# Autodesk Inventor assembly: ETrigger
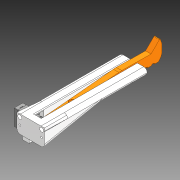
[picture p0: Inventor's stored thumbnail of the model, 180x180]
Saved by Autodesk Inventor 2020 (Build 240168000, 168)
## iProperties
Created: 2020-09-14
Part Number: ETrigger
Document SubType Name: Assembly
Designer: DDeGo
Author: DDeGo
Revision Number: PRODUCT_VERSION_IDPRODUCT_VERSION_DESCR
## Documents named in this file (4)
- C:\Users\DDeGo\Documents\Drew\Projects\Nerf Aim Assist\ESPER\ETrigger.iam
- C:\Users\DDeGo\Documents\Drew\Projects\Nerf Aim Assist\ESPER\SearE.ipt
- C:\Users\DDeGo\Documents\Drew\Projects\Nerf Aim Assist\ESPER\ETriggerGrip.ipt
- C:\Users\DDeGo\Documents\Drew\Projects\Nerf Aim Assist\Cad\MG90servo_body.ipt
## Components (3 placed, 3 different names)
1. NAUO_ID19 — Mate:1, Mate:2
2. ETriggerGrip:1 — Mate:1, Mate:2, Mate:3, Angle:1, Mate:4
3. MG90servo_body:1 — Mate:3, Angle:1, Mate:4
## Relationships (5: Mate 4, Angle 1)
- Mate:1: NAUO_ID19 ↔ ETriggerGrip:1
- Mate:2 (0.5 mm): NAUO_ID19 ↔ ETriggerGrip:1
- Mate:3: ETriggerGrip:1 ↔ MG90servo_body:1
- Angle:1 (180 deg): ETriggerGrip:1 ↔ MG90servo_body:1
- Mate:4: ETriggerGrip:1 ↔ MG90servo_body:1
